# Autodesk Inventor assembly: 足首_1_MIR
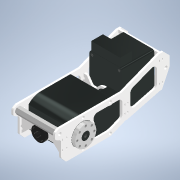
[picture p0: Inventor's stored thumbnail of the model, 180x180]
Saved by Autodesk Inventor 2020 (Build 240168000, 168)
## iProperties
Created: 2016-04-27
Part Number: 足首_1_MIR
Document SubType Name: Assembly
Designer: masato
Mass: 229.672 g
Surface Area: 385.784 cm^2
Volume: 116.119 cm^3
Density: 1.97789 g/cm^3
Author: hiroaki
## Documents named in this file (10)
- C:\Users\naoki\Documents\Inventor\CitBrains\git_clone\OpenPlatform167\付け根再設計1\OpenPlatform_ver3_0\下半身\足首\足首_1_MIR.iam
- C:\Users\naoki\Documents\Inventor\CitBrains\git_clone\OpenPlatform167\付け根再設計1\OpenPlatform_ver3_0\既製品\B3M11xx.ipt
- C:\Users\naoki\Documents\Inventor\CitBrains\git_clone\OpenPlatform167\付け根再設計1\OpenPlatform_ver3_0\既製品\B3M10xx.ipt
- C:\Users\naoki\Documents\Inventor\CitBrains\git_clone\OpenPlatform167\付け根再設計1\OpenPlatform_ver3_0\既製品\free_horn.ipt
- C:\Users\naoki\Documents\Inventor\CitBrains\git_clone\OpenPlatform167\付け根再設計1\OpenPlatform_ver3_0\下半身\足首\足首_メインフレーム_1_1.ipt
- C:\Users\naoki\Documents\Inventor\CitBrains\git_clone\OpenPlatform167\付け根再設計1\OpenPlatform_ver3_0\下半身\足首\足首_サブフレーム_1_1.ipt
- C:\Users\naoki\Documents\Inventor\CitBrains\git_clone\OpenPlatform167\付け根再設計1\OpenPlatform_ver3_0\下半身\足首\足首_サブフレーム_1_2.ipt
- C:\Users\naoki\Documents\Inventor\CitBrains\git_clone\OpenPlatform167\付け根再設計1\OpenPlatform_ver3_0\下半身\足首\足首_サブフレーム_1_3.ipt
- C:\Users\naoki\Documents\Inventor\CitBrains\git_clone\OpenPlatform167\付け根再設計1\OpenPlatform_ver3_0\下半身_160823\付け根\付け根_サブフレーム_1_4.ipt
- C:\Users\naoki\Documents\Inventor\CitBrains\git_clone\OpenPlatform167\付け根再設計1\OpenPlatform_ver3_0\既製品\SLSBF6-39_5-M3-N3.ipt
## Components (11 placed, 8 different names)
1. B3M11xx:1 — 挿入:23, 挿入:27, 挿入:26, 挿入:25, 挿入:24, 挿入:53, 挿入:52, 挿入:51, 挿入:36
2. B3M11xx:2 — 挿入:44, 挿入:43
3. free_horn:1 — 挿入:23
4. 足首_メインフレーム_1_1:1 — 挿入:27, 挿入:26, 挿入:25, 挿入:24, メイト:2, メイト:1, メイト:3, メイト:6, メイト:5, メイト:4, メイト:8, 挿入:54, 挿入:55
5. 足首_メインフレーム_1_1:2 — 挿入:53, 挿入:52, 挿入:51, 挿入:36, メイト:10, メイト:9
6. 足首_サブフレーム_1_1:1 — メイト:2, メイト:1, メイト:3
7. 足首_サブフレーム_1_2:1 — メイト:6, メイト:5, メイト:4, 挿入:44, 挿入:43
8. 足首_サブフレーム_1_3:1 — メイト:10, メイト:9, メイト:8, 挿入:50
9. 付け根_サブフレーム_1_4:1 — 挿入:50
10. SLSBF6-39_5-M3-N3:1 — 挿入:54
11. SLSBF6-39_5-M3-N3:2 — 挿入:55
## Relationships (23: Insert 14, Mate 9)
- 挿入:23 [Insert] (0.2 mm): B3M11xx:1 ↔ free_horn:1
- 挿入:27 [Insert]: B3M11xx:1 ↔ 足首_メインフレーム_1_1:1
- 挿入:26 [Insert]: B3M11xx:1 ↔ 足首_メインフレーム_1_1:1
- 挿入:25 [Insert]: B3M11xx:1 ↔ 足首_メインフレーム_1_1:1
- 挿入:24 [Insert]: B3M11xx:1 ↔ 足首_メインフレーム_1_1:1
- メイト:2 [Mate]: 足首_メインフレーム_1_1:1 ↔ 足首_サブフレーム_1_1:1
- メイト:1 [Mate] (0.01 mm): 足首_メインフレーム_1_1:1 ↔ 足首_サブフレーム_1_1:1
- メイト:3 [Mate] (0.01 mm): 足首_メインフレーム_1_1:1 ↔ 足首_サブフレーム_1_1:1
- メイト:6 [Mate] (0.01 mm): 足首_メインフレーム_1_1:1 ↔ 足首_サブフレーム_1_2:1
- メイト:5 [Mate] (0.01 mm): 足首_メインフレーム_1_1:1 ↔ 足首_サブフレーム_1_2:1
- メイト:4 [Mate]: 足首_メインフレーム_1_1:1 ↔ 足首_サブフレーム_1_2:1
- 挿入:53 [Insert]: B3M11xx:1 ↔ 足首_メインフレーム_1_1:2
- 挿入:52 [Insert]: B3M11xx:1 ↔ 足首_メインフレーム_1_1:2
- 挿入:51 [Insert]: B3M11xx:1 ↔ 足首_メインフレーム_1_1:2
- 挿入:36 [Insert]: B3M11xx:1 ↔ 足首_メインフレーム_1_1:2
- メイト:10 [Mate] (0.01 mm): 足首_メインフレーム_1_1:2 ↔ 足首_サブフレーム_1_3:1
- メイト:9 [Mate] (0.01 mm): 足首_メインフレーム_1_1:2 ↔ 足首_サブフレーム_1_3:1
- メイト:8 [Mate]: 足首_メインフレーム_1_1:1 ↔ 足首_サブフレーム_1_3:1
- 挿入:44 [Insert]: B3M11xx:2 ↔ 足首_サブフレーム_1_2:1
- 挿入:43 [Insert]: B3M11xx:2 ↔ 足首_サブフレーム_1_2:1
- 挿入:50 [Insert]: 足首_サブフレーム_1_3:1 ↔ 付け根_サブフレーム_1_4:1
- 挿入:54 [Insert]: 足首_メインフレーム_1_1:1 ↔ SLSBF6-39_5-M3-N3:1
- 挿入:55 [Insert]: 足首_メインフレーム_1_1:1 ↔ SLSBF6-39_5-M3-N3:2
